# Autodesk Inventor assembly: Ensamblaje1
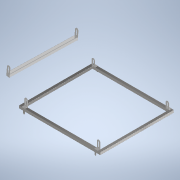
[picture p0: Inventor's stored thumbnail of the model, 180x180]
Saved by Autodesk Inventor 2021 (Build 250183000, 183)
## iProperties
Created: 2022-09-12
Part Number: Ensamblaje1
Document SubType Name: Conjunto soldado
Designer: arthu
Weld Material: Acero, fundido
Author: arthu
## Documents named in this file (5)
- C:\Users\arthu\Desktop\TersusMax\Diseño_2022\Ensamblaje1.iam
- C:\Users\arthu\Desktop\TersusMax\Diseño_2022\Pieza3.ipt
- C:\Users\arthu\Desktop\TersusMax\Diseño_2022\Pieza4.ipt
- C:\Users\arthu\Desktop\TersusMax\Diseño_2022\Pieza5.ipt
- C:\Users\arthu\Desktop\TersusMax\Diseño_2022\Pieza6.ipt
## Components (8 placed, 4 different names)
1. Pieza3:1 — De rotación:1, Rígido:1, De rotación:2, Rígido:2, De rotación:3
2. Pieza4:1 — Rígido:2, De rotación:3
3. Pieza4:2 — De rotación:2
4. Pieza4:3 — Rígido:1
5. Pieza4:4 — De rotación:1
6. Pieza5:1 — Rígido:3, Rígido:4
7. Pieza6:1 — Rígido:3
8. Pieza6:2 — Rígido:4
## Relationships (7: WeldJoint 4, RevoluteJoint 3)
- De rotación:1 [RevoluteJoint]: Pieza3:1 ↔ Pieza4:4
- Rígido:1 [WeldJoint]: Pieza3:1 ↔ Pieza4:3
- De rotación:2 [RevoluteJoint]: Pieza3:1 ↔ Pieza4:2
- Rígido:2 [WeldJoint]: Pieza3:1 ↔ Pieza4:1
- De rotación:3 [RevoluteJoint]: Pieza3:1 ↔ Pieza4:1
- Rígido:3 [WeldJoint]: Pieza5:1 ↔ Pieza6:1
- Rígido:4 [WeldJoint]: Pieza5:1 ↔ Pieza6:2
